# Autodesk Inventor assembly: MK5n, A (2)
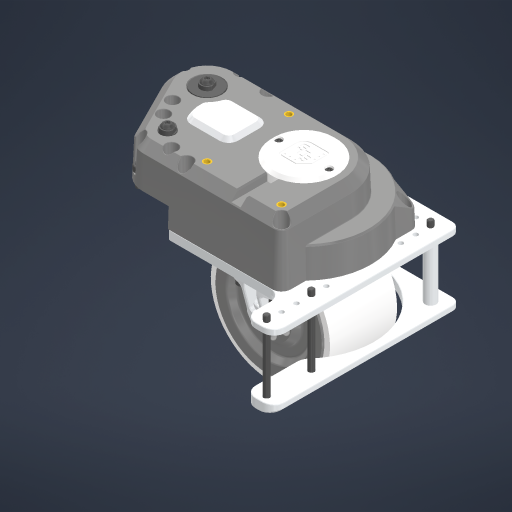
[picture p0: Inventor's stored thumbnail of the model, 512x512]
Saved by Autodesk Inventor 2024.4 (Build 284460000, 460)
## iProperties
Created: 2026-01-06
Part Number: MK5n, A (2)
Document SubType Name: Assembly
Designer: Kenji
Mass: 1769.01 g
Surface Area: 2127.48 cm^2
Volume: 1270.46 cm^3
Density: 1.39242 g/cm^3
Author: Kenji
Sending System: SOLIDWORKS 2022-2022290
MC: AMD64
MC_MODEL: Intel64 Family 6 Model 158 Stepping 10, GenuineIntel
OS: Windows_NT
FRU: Parasolid Version 33.1, build 260,  4-25-2022
FORMAT: text
GUISE: transmit
KEY: FILEMK5n, A.x_t
DATE: Fri Aug  8 12:42:24 2025
## Documents named in this file (11)
- C:\Users\Kenji\Documents\GitHub\1622-2026-Rebuilt\COTS Library\MK5n, A (2).iam
- C:\Users\Kenji\Downloads\MK5n, A (2)\MK5n, A (2)\MK5n, A (2).ipt
- C:\Users\Kenji\Downloads\MK5n, A (2)\MK5n, A (2)\MK5n, A (2)_1.ipt
- C:\Users\Kenji\Downloads\MK5n, A (2)\MK5n, A (2)\MK5n, A (2)_2.ipt
- C:\Users\Kenji\Downloads\MK5n, A (2)\MK5n, A (2)\MK5n, A (2)_3.ipt
- C:\Users\Kenji\Downloads\MK5n, A (2)\MK5n, A (2)\MK5n, A (2)_4.ipt
- C:\Users\Kenji\Downloads\MK5n, A (2)\MK5n, A (2)\MK5n, A (2)_5.ipt
- C:\Users\Kenji\Downloads\MK5n, A (2)\MK5n, A (2)\MK5n, A (2)_6.ipt
- C:\Users\Kenji\Downloads\MK5n, A (2)\MK5n, A (2)\MK5n, A (2)_7.ipt
- C:\Users\Kenji\Downloads\MK5n, A (2)\MK5n, A (2)\MK5n, A (2)_8.ipt
- C:\Users\Kenji\Downloads\MK5n, A (2)\MK5n, A (2)\MK5n, A (2)_9.ipt
## Components (10 placed, 10 different names)
1. MK5n, A (2) — Mate:1, Mate:2, Mate:3, Mate:4
2. MK5n, A (2)_1 — Mate:1, Mate:2, Angle:1
3. MK5n, A (2)_2 — Mate:5, Mate:8, Mate:9, Mate:10, Mate:11, Mate:12, Mate:13, Mate:14, Mate:15, Mate:16
4. MK5n, A (2)_3 — Mate:10, Mate:11
5. MK5n, A (2)_4 — Mate:12, Flush:2, Flush:3
6. MK5n, A (2)_5 — Mate:13, Flush:3, Mate:16
7. MK5n, A (2)_6 — Mate:14, Flush:1
8. MK5n, A (2)_7 — Mate:15, Flush:1, Flush:2
9. MK5n, A (2)_8 — Mate:6, Mate:7, Mate:8, Mate:9
10. MK5n, A (2)_9 — Mate:3, Mate:4, Angle:1, Mate:5, Mate:6, Mate:7
## Relationships (20: Mate 16, Flush 3, Angle 1)
- Mate:1: MK5n, A (2) ↔ MK5n, A (2)_1
- Mate:2: MK5n, A (2) ↔ MK5n, A (2)_1
- Mate:3: MK5n, A (2) ↔ MK5n, A (2)_9
- Mate:4: MK5n, A (2) ↔ MK5n, A (2)_9
- Angle:1 (0 deg): MK5n, A (2)_1 ↔ MK5n, A (2)_9
- Mate:5: MK5n, A (2)_2 ↔ MK5n, A (2)_9
- Mate:6: MK5n, A (2)_8 ↔ MK5n, A (2)_9
- Mate:7: MK5n, A (2)_8 ↔ MK5n, A (2)_9
- Mate:8: MK5n, A (2)_2 ↔ MK5n, A (2)_8
- Mate:9: MK5n, A (2)_2 ↔ MK5n, A (2)_8
- Mate:10: MK5n, A (2)_2 ↔ MK5n, A (2)_3
- Mate:11: MK5n, A (2)_2 ↔ MK5n, A (2)_3
- Mate:12: MK5n, A (2)_2 ↔ MK5n, A (2)_4
- Mate:13: MK5n, A (2)_2 ↔ MK5n, A (2)_5
- Mate:14: MK5n, A (2)_2 ↔ MK5n, A (2)_6
- Mate:15: MK5n, A (2)_2 ↔ MK5n, A (2)_7
- Flush:1: MK5n, A (2)_6 ↔ MK5n, A (2)_7
- Flush:2: MK5n, A (2)_4 ↔ MK5n, A (2)_7
- Flush:3: MK5n, A (2)_4 ↔ MK5n, A (2)_5
- Mate:16: MK5n, A (2)_2 ↔ MK5n, A (2)_5
